# Autodesk Inventor assembly: Assembly-payload-part1_tip_plate
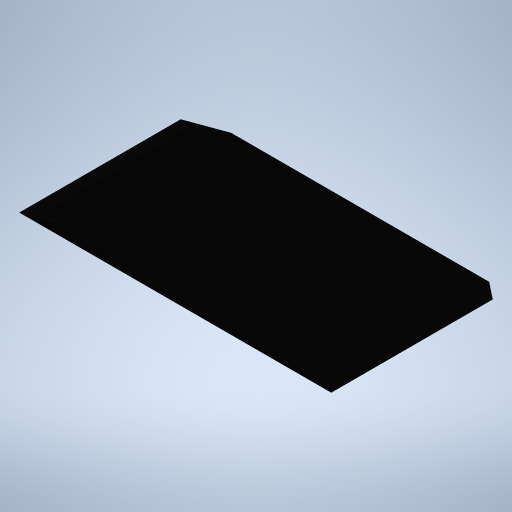
[picture p0: Inventor's stored thumbnail of the model, 512x512]
Saved by Autodesk Inventor 2023 (Build 270158000, 158)
## iProperties
Created: 2023-04-18
Part Number: Assembly-payload-part1_tip_plate
Document SubType Name: Assembly
Designer: ASARe-DAQ-PC
Author: ASARe-DAQ-PC
## Documents named in this file (2)
- D:\EB camera\model of EB camera\for manufacture\Assembly-payload-part1_tip_plate.iam
- D:\EB camera\model of EB camera\for manufacture\Model Shell_part1_tip_plate.ipt
## Components (1 placed, 1 different names)
1. Model Shell_part1_tip_plate:1 — Mate:1
## Relationships (1: Mate 1)
- Mate:1: Model Shell_part1_tip_plate:1
